# Autodesk Inventor assembly: case_assembly
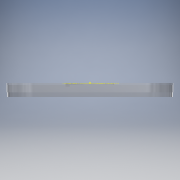
[picture p0: Inventor's stored thumbnail of the model, 180x180]
Saved by Autodesk Inventor 2019 (Build 230136000, 136)
## iProperties
Created: 2019-01-02
Part Number: case_assembly
Document SubType Name: Assembly
Designer: jmc
Author: jmc
## Documents named in this file (12)
- C:\Users\l0086\Desktop\Models\CatFeeder\version2 (fixed enclosure)\version2_newcone.iam
- C:\Users\l0086\Desktop\Models\CatFeeder\Case\version2\case.ipt
- C:\Users\l0086\Desktop\Models\3party\Boards\ArduinoNano\arduino nano.iam
- C:\Users\l0086\Desktop\Models\3party\Boards\Raspberry Pi 3\Raspberry Pi 3.ipt
- C:\Users\l0086\Desktop\Models\3party\Trasformer\Transformer.ipt
- C:\Users\l0086\Desktop\Models\CatFeeder\Case\version2\case_top.ipt
- C:\Users\l0086\Desktop\Models\CatFeeder\Case\version2\case_bottom.ipt
- C:\Users\l0086\Desktop\Models\CatFeeder\Case\version2\Pata.ipt
- C:\Users\l0086\Desktop\Models\CatFeeder\Case\version2\pata_macho.ipt
- C:\Users\l0086\Desktop\Models\CatFeeder\JarCone\version2\cono_nuevo.ipt
- C:\Users\l0086\Desktop\Models\CatFeeder\JarCone\version2\adaptador_cono.ipt
- C:\Users\l0086\Desktop\Models\CatFeeder\Jar\Jar.ipt
## Components (17 placed, 11 different names)
1. case:1
2. case_top:1 — Rigid:9, Rigid:10, Flush:2
3. cono_nuevo:1 — Rigid:11, Rigid:12
4. adaptador_cono:1 — Rigid:10, Rigid:11, Flush:2
5. Jar:1 — Rigid:12
6. case_bottom:1 — Rigid:1, Rigid:3, Rigid:4, Flush:1, Rotational:1, Rigid:6, Rigid:7, Rigid:8, Rigid:9
7. arduino nano:1 [sub-assembly] — Rigid:4
8. Raspberry Pi 3:1 — Rigid:1
9. Transformer:1 — Rigid:3
10. pata_macho:4 — Rotational:5
11. pata_macho:3 — Rotational:3
12. pata_macho:2 — Rotational:4
13. pata_macho:1 — Rotational:2
14. Pata:1 — Flush:1, Rotational:1, Rotational:2
15. Pata:2 — Rigid:8, Rotational:5
16. Pata:3 — Rigid:7, Rotational:3
17. Pata:4 — Rigid:6, Rotational:4
## Relationships (17: WeldJoint 10, RevoluteJoint 5, Flush 2)
- Rigid:1 [WeldJoint]: case_bottom:1 ↔ Raspberry Pi 3:1
- Rigid:3 [WeldJoint]: case_bottom:1 ↔ Transformer:1
- Rigid:4 [WeldJoint]: case_bottom:1 ↔ arduino nano:1
- Flush:1: case_bottom:1 ↔ Pata:1
- Rotational:1 [RevoluteJoint]: case_bottom:1 ↔ Pata:1
- Rigid:6 [WeldJoint]: case_bottom:1 ↔ Pata:4
- Rigid:7 [WeldJoint]: case_bottom:1 ↔ Pata:3
- Rigid:8 [WeldJoint]: case_bottom:1 ↔ Pata:2
- Rotational:2 [RevoluteJoint]: pata_macho:1 ↔ Pata:1
- Rotational:3 [RevoluteJoint]: pata_macho:3 ↔ Pata:3
- Rotational:4 [RevoluteJoint]: pata_macho:2 ↔ Pata:4
- Rotational:5 [RevoluteJoint]: pata_macho:4 ↔ Pata:2
- Rigid:9 [WeldJoint]: case_top:1 ↔ case_bottom:1
- Rigid:10 [WeldJoint]: case_top:1 ↔ adaptador_cono:1
- Rigid:11 [WeldJoint]: cono_nuevo:1 ↔ adaptador_cono:1
- Rigid:12 [WeldJoint]: cono_nuevo:1 ↔ Jar:1
- Flush:2: case_top:1 ↔ adaptador_cono:1
## Named parameters: HOLE_TOLERANCE = 0.15 mm, CASE_TOLERANCE = 0.08 mm
